# Autodesk Inventor assembly: l-holder_2020-asm
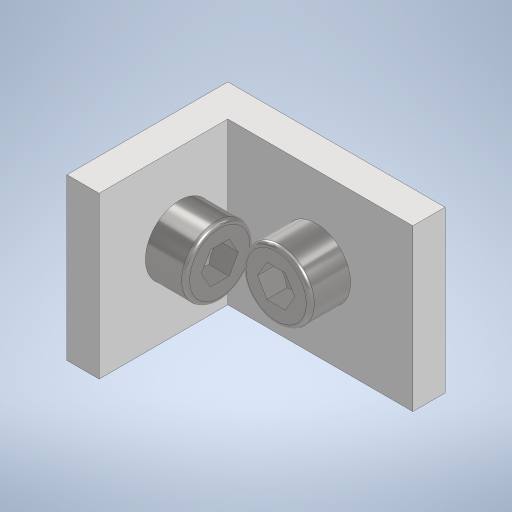
[picture p0: Inventor's stored thumbnail of the model, 512x512]
Saved by Autodesk Inventor 2024 (Build 280153000, 153)
## iProperties
Created: 2025-12-26
Part Number: l-holder_2020-asm
Document SubType Name: Assembly
Designer: schar
Author: schar
## Documents named in this file (4)
- C:\Users\schar\Desktop\projectBlueprint\AMSTS\hardware\l-holder_2020-asm.iam
- C:\Users\schar\Desktop\projectBlueprint\AMSTS\hardware\l-holder_2020.ipt
- C:\Users\schar\Desktop\projectBlueprint\AMSTS\hardware\tnut_m5_2020.ipt
- C:\Users\schar\Documents\Inventor\Content Center Files\R2024\en-US\ISO 4762(1)\DIN EN ISO 4762 - M5 x 10.ipt
## Components (5 placed, 3 different names)
1. l-holder_2020:1 — Rigid:1, Rigid:2, Mate:1, Mate:2, Mate:3, Mate:4
2. tnut_m5_2020:1 — Rigid:1
3. tnut_m5_2020:2 — Rigid:2
4. DIN EN ISO 4762 M5 x 10:1 — Mate:2, Mate:3
5. DIN EN ISO 4762 M5 x 10:2 — Mate:1, Mate:4
## Relationships (6: Mate 4, WeldJoint 2)
- Rigid:1 [WeldJoint] (-0.159 mm): l-holder_2020:1 ↔ tnut_m5_2020:1
- Rigid:2 [WeldJoint] (-0.159 mm): l-holder_2020:1 ↔ tnut_m5_2020:2
- Mate:1: l-holder_2020:1 ↔ DIN EN ISO 4762 M5 x 10:2
- Mate:2: l-holder_2020:1 ↔ DIN EN ISO 4762 M5 x 10:1
- Mate:3: l-holder_2020:1 ↔ DIN EN ISO 4762 M5 x 10:1
- Mate:4: l-holder_2020:1 ↔ DIN EN ISO 4762 M5 x 10:2
